# Autodesk Inventor assembly: Schaal test met -alles-
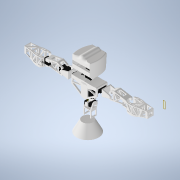
[picture p0: Inventor's stored thumbnail of the model, 180x180]
Saved by Autodesk Inventor 2022 (Build 260153000, 153)
## iProperties
Created: 2022-04-29
Part Number: Schaal test met -alles-
Document SubType Name: Assembly
Designer: kajve
Author: kajve
## Documents named in this file (10)
- C:\Users\kajve\OneDrive\Documenten\GitHub\Arny-de-humanoid-robot\Parts\Tests\Schaal test met -alles-.iam
- C:\Users\kajve\OneDrive\Documenten\GitHub\Arny-de-humanoid-robot\Parts\Torso.ipt
- C:\Users\kajve\OneDrive\Documenten\GitHub\Arny-de-humanoid-robot\Parts\Tests\Arms-with-motor.iam
- C:\Users\kajve\OneDrive\Documenten\GitHub\Arny-de-humanoid-robot\Parts\Tests\Spine test.iam
- C:\Users\kajve\OneDrive\Documenten\GitHub\Arny-de-humanoid-robot\Parts\Spine.ipt
- C:\Users\kajve\OneDrive\Documenten\GitHub\Arny-de-humanoid-robot\Parts\Imported Components\SERVO motor\Axel Mount.ipt
- C:\Users\kajve\OneDrive\Documenten\GitHub\Arny-de-humanoid-robot\Parts\Tests\Nek met hoofd.iam
- C:\Users\kajve\OneDrive\Documenten\GitHub\Arny-de-humanoid-robot\Parts\Tests\Arms-with-motor-mirrored.iam
- C:\Users\kajve\OneDrive\Documenten\GitHub\Arny-de-humanoid-robot\Parts\Basis (WIP).ipt
- C:\Users\kajve\OneDrive\Documenten\GitHub\Arny-de-humanoid-robot\Parts\Imported Components\SERVO motor\Servo MOtor.ipt
## Components (10 placed, 9 different names)
1. Torso:1 — Mate:4, Mate:5, Flush:4, Mate:6, Mate:7, Mate:8, Mate:9, Mate:10, Mate:11
2. Arms-with-motor:2 [sub-assembly]
3. Spine test:1 [sub-assembly] — Mate:3, Flush:2, Flush:3
4. Spine:1 — Mate:1, Mate:2, Flush:1, Flush:2, Flush:3
5. Axel Mount:1 — Mate:1, Mate:2, Flush:1, Mate:3
6. Nek met hoofd:1 [sub-assembly] — Mate:4, Mate:5, Flush:4
7. Arms-with-motor-mirrored:1 [sub-assembly]
8. Basis (WIP):1
9. Servo MOtor:1 — Mate:6, Mate:7, Mate:8
10. Servo MOtor:2 — Mate:9, Mate:10, Mate:11
## Relationships (15: Mate 11, Flush 4)
- Mate:1: Spine:1 ↔ Axel Mount:1
- Mate:2: Spine:1 ↔ Axel Mount:1
- Flush:1: Spine:1 ↔ Axel Mount:1
- Mate:3 (-4.8 mm): Spine test:1 ↔ Axel Mount:1
- Flush:2 (-7.8 mm): Spine test:1 ↔ Spine:1
- Flush:3 (-26 mm): Spine test:1 ↔ Spine:1
- Mate:4: Torso:1 ↔ Nek met hoofd:1
- Mate:5: Torso:1 ↔ Nek met hoofd:1
- Flush:4: Torso:1 ↔ Nek met hoofd:1
- Mate:6: Torso:1 ↔ Servo MOtor:1
- Mate:7: Torso:1 ↔ Servo MOtor:1
- Mate:8: Torso:1 ↔ Servo MOtor:1
- Mate:9: Torso:1 ↔ Servo MOtor:2
- Mate:10: Torso:1 ↔ Servo MOtor:2
- Mate:11: Torso:1 ↔ Servo MOtor:2
